# Autodesk Inventor assembly: D5_Assembly_3.0_wires_052225
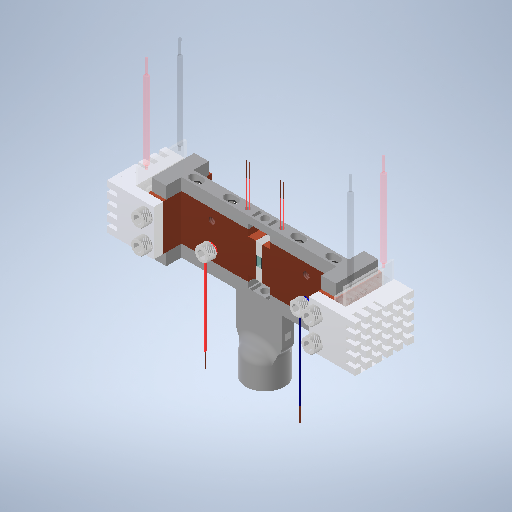
[picture p0: Inventor's stored thumbnail of the model, 512x512]
Saved by Autodesk Inventor 2025 (Build 290162000, 162)
## iProperties
Created: 2024-04-25
Part Number: D5_Assembly_3.0_wires_052225
Document SubType Name: Assembly
Designer: warke
Author: warke
## Documents named in this file (21)
- G:\Shared drives\Kerlin lab shared\Users\ChrisW\EOD\Builds\reload_mount_1p2\D5_Assembly_3.0_wires_052225.iam
- G:\Shared drives\Kerlin lab shared\Users\ChrisW\EOD\Builds\reload_mount_1p2\copper_thermal_contact.ipt
- G:\Shared drives\Kerlin lab shared\Users\ChrisW\EOD\Builds\reload_mount_1p2\AlN_thermal_contact.ipt
- G:\Shared drives\Kerlin lab shared\Users\ChrisW\EOD\Builds\reload_mount_1p2\KTN_Chip_4mmX3p2mmX1p2mm.ipt
- G:\Shared drives\Kerlin lab shared\Users\ChrisW\EOD\Builds\reload_mount_1p2\TEC3-2.5-Solidworks (1).ipt
- G:\Shared drives\Kerlin lab shared\Users\ChrisW\EOD\Builds\reload_mount_1p2\Al_tec_holder.ipt
- G:\Shared drives\Kerlin lab shared\Users\ChrisW\EOD\Builds\reload_mount_1p2\92196A052_18-8 Stainless Steel Socket Head Screw.ipt
- G:\Shared drives\Kerlin lab shared\Users\ChrisW\EOD\Builds\reload_mount_1p2\acrylic_temp_holder.ipt
- G:\Shared drives\Kerlin lab shared\Users\ChrisW\EOD\Builds\reload_mount_1p2\acrylic_side_holder_plunger2.ipt
- G:\Shared drives\Kerlin lab shared\Users\ChrisW\EOD\Builds\reload_mount_1p2\acrylic_side_holder_plunger_bottom.ipt
- G:\Shared drives\Kerlin lab shared\Users\ChrisW\EOD\Builds\reload_mount_1p2\acrylic_side_holder_plunger_top_keep.ipt
- G:\Shared drives\Kerlin lab shared\Users\ChrisW\EOD\Builds\reload_mount_1p2\graphite_new.ipt
- G:\Shared drives\Kerlin lab shared\Users\ChrisW\EOD\Builds\reload_mount_1p2\92196A951_18-8 Stainless Steel Socket Head Screw.ipt
- G:\Shared drives\Kerlin lab shared\Users\ChrisW\EOD\Builds\reload_mount_1p2\volt_screw_pneg.ipt
- G:\Shared drives\Kerlin lab shared\Users\ChrisW\EOD\Builds\reload_mount_1p2\volt_screw_pos.ipt
- \\134.84.4.92\general\engineering\3D_ReLOAD_2025\spacer1.ipt
- G:\Shared drives\Kerlin lab shared\Users\ChrisW\EOD\Builds\reload_mount_1p2\D5_Assembly_3.0_wires_052225\AIP\FEA\f2lulih1c.fins
- G:\Shared drives\Kerlin lab shared\Users\ChrisW\EOD\Builds\reload_mount_1p2\D5_Assembly_3.0_wires_052225\AIP\FEA\f2lulih1c.fsat
- G:\Shared drives\Kerlin lab shared\Users\ChrisW\EOD\Builds\reload_mount_1p2\D5_Assembly_3.0_wires_052225\AIP\FEA\f2lulih1c.ftes
- G:\Shared drives\Kerlin lab shared\Users\ChrisW\EOD\Builds\reload_mount_1p2\D5_Assembly_3.0_wires_052225\AIP\FEA\f2lulih1c.fwiz
- G:\Shared drives\Kerlin lab shared\Users\ChrisW\EOD\Builds\reload_mount_1p2\D5_Assembly_3.0_wires_052225\AIP\FEA\f2lulih40.fmsh
## Components (33 placed, 15 different names)
1. copper_thermal_contact:1 — Mate:14, Mate:15, Mate:18, Mate:19, Mate:22, Mate:23, Mate:68, Mate:70, Mate:77, Mate:78, Mate:79, Mate:80
2. copper_thermal_contact:2 — Mate:2, Mate:20, Mate:21, Mate:24, Mate:25, Mate:58, Mate:59, Mate:64, Mate:66, Mate:75, Mate:76, Mate:81, Mate:82
3. AlN_thermal_contact:2 — Mate:2, Mate:4, Mate:41, Mate:46, Mate:60, Flush:1
4. KTN_Chip_4mmX3p2mmX1p2mm:1 — Mate:4, Mate:32, Mate:45, Mate:47
5. Al_tec_holder:1 — Mate:63, Mate:65
6. Al_tec_holder:2 — Mate:14, Mate:15, Mate:67, Mate:69
7. 92196A052_18-8 Stainless Steel Socket Head Screw:1 — Mate:18
8. 92196A052_18-8 Stainless Steel Socket Head Screw:2 — Mate:19
9. 92196A052_18-8 Stainless Steel Socket Head Screw:3 — Mate:20
10. 92196A052_18-8 Stainless Steel Socket Head Screw:4 — Mate:21
11. 92196A052_18-8 Stainless Steel Socket Head Screw:5 — Mate:22
12. 92196A052_18-8 Stainless Steel Socket Head Screw:6 — Mate:23
13. 92196A052_18-8 Stainless Steel Socket Head Screw:7 — Mate:24
14. 92196A052_18-8 Stainless Steel Socket Head Screw:8 — Mate:25
15. acrylic_temp_holder:1 — Mate:32
16. acrylic_side_holder_plunger2:1 — Mate:41
17. acrylic_side_holder_plunger_bottom:1 — Mate:56, Mate:58, Mate:59, Mate:60, Mate:61, Angle:1, Angle:2
18. acrylic_side_holder_plunger_top_keep:1
19. AlN_thermal_contact:3 — Mate:45
20. graphite_new:1 — Mate:46
21. graphite_new:2 — Mate:47
22. 92196A052_18-8 Stainless Steel Socket Head Screw:10 — Mate:56
23. 92196A052_18-8 Stainless Steel Socket Head Screw:11 — Mate:61
24. 92196A951_18-8 Stainless Steel Socket Head Screw:1 — Mate:67, Mate:68
25. 92196A951_18-8 Stainless Steel Socket Head Screw:2 — Mate:65, Mate:66
26. 92196A951_18-8 Stainless Steel Socket Head Screw:3 — Mate:63, Mate:64
27. 92196A951_18-8 Stainless Steel Socket Head Screw:5 — Mate:69, Mate:70
28. 92196A951_18-8 Stainless Steel Socket Head Screw:6
29. TEC3-2.5-Solidworks (1):1 — Mate:75, Mate:76
30. TEC3-2.5-Solidworks (1):2 — Mate:77, Mate:78
31. volt_screw_pos:1 — Angle:1, Mate:79, Mate:80
32. volt_screw_pneg:1 — Angle:2, Mate:81, Mate:82
33. spacer1:1 — Flush:1
## Relationships (41: Mate 38, Angle 2, Flush 1)
- Mate:2: copper_thermal_contact:2 ↔ AlN_thermal_contact:2
- Mate:4: AlN_thermal_contact:2 ↔ KTN_Chip_4mmX3p2mmX1p2mm:1
- Mate:14: copper_thermal_contact:1 ↔ Al_tec_holder:2
- Mate:15: copper_thermal_contact:1 ↔ Al_tec_holder:2
- Mate:18: copper_thermal_contact:1 ↔ 92196A052_18-8 Stainless Steel Socket Head Screw:1
- Mate:19: copper_thermal_contact:1 ↔ 92196A052_18-8 Stainless Steel Socket Head Screw:2
- Mate:20: copper_thermal_contact:2 ↔ 92196A052_18-8 Stainless Steel Socket Head Screw:3
- Mate:21: copper_thermal_contact:2 ↔ 92196A052_18-8 Stainless Steel Socket Head Screw:4
- Mate:22: copper_thermal_contact:1 ↔ 92196A052_18-8 Stainless Steel Socket Head Screw:5
- Mate:23: copper_thermal_contact:1 ↔ 92196A052_18-8 Stainless Steel Socket Head Screw:6
- Mate:24: copper_thermal_contact:2 ↔ 92196A052_18-8 Stainless Steel Socket Head Screw:7
- Mate:25: copper_thermal_contact:2 ↔ 92196A052_18-8 Stainless Steel Socket Head Screw:8
- Mate:32: KTN_Chip_4mmX3p2mmX1p2mm:1 ↔ acrylic_temp_holder:1
- Mate:41: AlN_thermal_contact:2 ↔ acrylic_side_holder_plunger2:1
- Mate:45: KTN_Chip_4mmX3p2mmX1p2mm:1 ↔ AlN_thermal_contact:3
- Mate:46: AlN_thermal_contact:2 ↔ graphite_new:1
- Mate:47: KTN_Chip_4mmX3p2mmX1p2mm:1 ↔ graphite_new:2
- Mate:56: acrylic_side_holder_plunger_bottom:1 ↔ 92196A052_18-8 Stainless Steel Socket Head Screw:10
- Mate:58: copper_thermal_contact:2 ↔ acrylic_side_holder_plunger_bottom:1
- Mate:59: copper_thermal_contact:2 ↔ acrylic_side_holder_plunger_bottom:1
- Mate:60: AlN_thermal_contact:2 ↔ acrylic_side_holder_plunger_bottom:1
- Mate:61: acrylic_side_holder_plunger_bottom:1 ↔ 92196A052_18-8 Stainless Steel Socket Head Screw:11
- Mate:63: Al_tec_holder:1 ↔ 92196A951_18-8 Stainless Steel Socket Head Screw:3
- Mate:64: copper_thermal_contact:2 ↔ 92196A951_18-8 Stainless Steel Socket Head Screw:3
- Mate:65: Al_tec_holder:1 ↔ 92196A951_18-8 Stainless Steel Socket Head Screw:2
- Mate:66: copper_thermal_contact:2 ↔ 92196A951_18-8 Stainless Steel Socket Head Screw:2
- Mate:67: Al_tec_holder:2 ↔ 92196A951_18-8 Stainless Steel Socket Head Screw:1
- Mate:68: copper_thermal_contact:1 ↔ 92196A951_18-8 Stainless Steel Socket Head Screw:1
- Mate:69: Al_tec_holder:2 ↔ 92196A951_18-8 Stainless Steel Socket Head Screw:5
- Mate:70: copper_thermal_contact:1 ↔ 92196A951_18-8 Stainless Steel Socket Head Screw:5
- Mate:75: copper_thermal_contact:2 ↔ TEC3-2.5-Solidworks (1):1
- Mate:76: copper_thermal_contact:2 ↔ TEC3-2.5-Solidworks (1):1
- Mate:77: copper_thermal_contact:1 ↔ TEC3-2.5-Solidworks (1):2
- Mate:78: copper_thermal_contact:1 ↔ TEC3-2.5-Solidworks (1):2
- Angle:1 (0 deg): acrylic_side_holder_plunger_bottom:1 ↔ volt_screw_pos:1
- Angle:2 (0 deg): acrylic_side_holder_plunger_bottom:1 ↔ volt_screw_pneg:1
- Mate:79: copper_thermal_contact:1 ↔ volt_screw_pos:1
- Mate:80: copper_thermal_contact:1 ↔ volt_screw_pos:1
- Mate:81: copper_thermal_contact:2 ↔ volt_screw_pneg:1
- Mate:82: copper_thermal_contact:2 ↔ volt_screw_pneg:1
- Flush:1: AlN_thermal_contact:2 ↔ spacer1:1
## Named parameters: sa_0 = 177.929
note: some values were not read from the file. Shown as the stored number, unit unknown: "sa_0".
